# Autodesk Inventor assembly: axis5_6
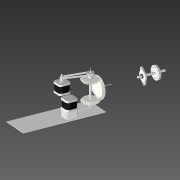
[picture p0: Inventor's stored thumbnail of the model, 180x180]
Saved by Autodesk Inventor 2020 (Build 240168000, 168)
## iProperties
Created: 2020-05-15
Part Number: axis5_6
Document SubType Name: Assembly
Designer: stefa
Author: stefa
## Documents named in this file (13)
- D:\github_gedeeld\BeerMinder\3D-model\axis5_6\axis5_6.iam
- D:\github_gedeeld\BeerMinder\3D-model\pulleys\tandriem32Tnaar16T_lengte240.ipt
- D:\github_gedeeld\BeerMinder\3D-model\pulleys\GT2 Timing Pulley 36T - 8mm as.ipt
- D:\github_gedeeld\BeerMinder\3D-model\stepper motors\42BYG Stepper Motor.ipt
- D:\github_gedeeld\BeerMinder\3D-model\pulleys\GT2 Pulley 16T - 5mm as.ipt
- D:\github_gedeeld\BeerMinder\3D-model\axis5_6\as_d8_l100.ipt
- D:\github_gedeeld\BeerMinder\3D-model\axis5_6\axis5_6\Design Accelerator\Bevel Gears1.iam
- D:\github_gedeeld\BeerMinder\3D-model\axis5_6\endeffector mount part.ipt
- D:\github_gedeeld\BeerMinder\3D-model\axis5_6\bovenarm - links.ipt
- D:\github_gedeeld\BeerMinder\3D-model\axis5_6\as naar endeffector.ipt
- D:\github_gedeeld\BeerMinder\3D-model\axis5_6\stepper spacer.ipt
- D:\github_gedeeld\BeerMinder\3D-model\axis5_6\axis5_6\Design Accelerator\Bevel Gear11.ipt
- D:\github_gedeeld\BeerMinder\3D-model\bearings\bloklager.ipt
## Components (16 placed, 12 different names)
1. tandriem32Tnaar16T_lengte240:1 — Mate:5, Mate:6, Mate:57, Mate:58
2. GT2 Pulley 16T - 5mm as:1 — Mate:5, Mate:6, Mate:51, Mate:53
3. as_d8_l100:1 — Mate:26, Flush:2, Mate:40, Mate:41, Mate:50, Mate:56
4. tandriem32Tnaar16T_lengte240:2 — Mate:44, Mate:46, Mate:48, Mate:49
5. Bevel Gears:1 [sub-assembly] — Mate:26, Mate:28, Mate:38, Mate:39
6. 42BYG Stepper Motor:2 — Flush:1, Mate:19, Mate:32, Angle:2, Mate:33, Mate:35, Mate:36, Mate:37, Mate:51, Mate:53, Mate:54, Mate:55
7. 42BYG Stepper Motor:3 — Flush:1, Mate:19, Angle:1, Mate:45, Mate:47, Mate:54, Mate:55
8. endeffector mount part:1 — Mate:27
9. bovenarm - links:1 — Mate:32, Angle:2, Mate:33, Angle:3, Mate:34, Mate:40, Mate:41
10. as naar endeffector:1 — Mate:27, Mate:28, Mate:29, Mate:30, Mate:31, Angle:1, Mate:42
11. stepper spacer:1 — Mate:34, Mate:35, Mate:36, Mate:37
12. Bevel Gear1:1 — Mate:38, Mate:39
13. bloklager:1 — Mate:42
14. GT2 Pulley 16T - 5mm as:2 — Mate:44, Mate:45, Mate:46, Mate:47
15. GT2 Timing Pulley 36T - 8mm as:5 — Mate:48, Mate:49, Mate:50
16. GT2 Timing Pulley 36T - 8mm as:6 — Mate:56, Mate:57, Mate:58
## Relationships (39: Mate 34, Angle 3, Flush 2)
- Mate:5: tandriem32Tnaar16T_lengte240:1 ↔ GT2 Pulley 16T - 5mm as:1
- Mate:6 (0.5 mm): tandriem32Tnaar16T_lengte240:1 ↔ GT2 Pulley 16T - 5mm as:1
- Flush:1: 42BYG Stepper Motor:2 ↔ 42BYG Stepper Motor:3
- Mate:19 (2 mm): 42BYG Stepper Motor:2 ↔ 42BYG Stepper Motor:3
- Mate:26: as_d8_l100:1 ↔ Bevel Gears:1
- Mate:27: endeffector mount part:1 ↔ as naar endeffector:1
- Mate:28: Bevel Gears:1 ↔ as naar endeffector:1
- Mate:29: as naar endeffector:1
- Mate:30: as naar endeffector:1
- Mate:31: as naar endeffector:1
- Angle:1 (0 deg): 42BYG Stepper Motor:3 ↔ as naar endeffector:1
- Mate:32: 42BYG Stepper Motor:2 ↔ bovenarm - links:1
- Angle:2 (0 deg): 42BYG Stepper Motor:2 ↔ bovenarm - links:1
- Mate:33: 42BYG Stepper Motor:2 ↔ bovenarm - links:1
- Angle:3 (0 deg): bovenarm - links:1
- Mate:34: bovenarm - links:1 ↔ stepper spacer:1
- Mate:35: 42BYG Stepper Motor:2 ↔ stepper spacer:1
- Mate:36: 42BYG Stepper Motor:2 ↔ stepper spacer:1
- Mate:37: 42BYG Stepper Motor:2 ↔ stepper spacer:1
- Mate:38: Bevel Gears:1 ↔ Bevel Gear1:1
- Mate:39 (26.661 mm): Bevel Gears:1 ↔ Bevel Gear1:1
- Flush:2: as_d8_l100:1
- Mate:40: as_d8_l100:1 ↔ bovenarm - links:1
- Mate:41: as_d8_l100:1 ↔ bovenarm - links:1
- Mate:42: as naar endeffector:1 ↔ bloklager:1
- Mate:44: tandriem32Tnaar16T_lengte240:2 ↔ GT2 Pulley 16T - 5mm as:2
- Mate:45: 42BYG Stepper Motor:3 ↔ GT2 Pulley 16T - 5mm as:2
- Mate:46 (0.5 mm): tandriem32Tnaar16T_lengte240:2 ↔ GT2 Pulley 16T - 5mm as:2
- Mate:47 (1 mm): 42BYG Stepper Motor:3 ↔ GT2 Pulley 16T - 5mm as:2
- Mate:48: tandriem32Tnaar16T_lengte240:2 ↔ GT2 Timing Pulley 36T - 8mm as:5
- Mate:49 (0.5 mm): tandriem32Tnaar16T_lengte240:2 ↔ GT2 Timing Pulley 36T - 8mm as:5
- Mate:50: as_d8_l100:1 ↔ GT2 Timing Pulley 36T - 8mm as:5
- Mate:51: GT2 Pulley 16T - 5mm as:1 ↔ 42BYG Stepper Motor:2
- Mate:53 (1 mm): GT2 Pulley 16T - 5mm as:1 ↔ 42BYG Stepper Motor:2
- Mate:54: 42BYG Stepper Motor:2 ↔ 42BYG Stepper Motor:3
- Mate:55: 42BYG Stepper Motor:2 ↔ 42BYG Stepper Motor:3
- Mate:56: as_d8_l100:1 ↔ GT2 Timing Pulley 36T - 8mm as:6
- Mate:57 (0.5 mm): tandriem32Tnaar16T_lengte240:1 ↔ GT2 Timing Pulley 36T - 8mm as:6
- Mate:58: tandriem32Tnaar16T_lengte240:1 ↔ GT2 Timing Pulley 36T - 8mm as:6
